# Autodesk Inventor assembly: Toughbox Nano Long Hex Output Shaft
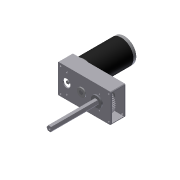
[picture p0: Inventor's stored thumbnail of the model, 180x180]
Saved by Autodesk Inventor 2013 (Build 170138000, 138)
## iProperties
Created: 2012-06-03
Part Number: Toughbox Nano Long Hex Output Shaft
Document SubType Name: Assembly
Designer: Nemo
Author: Nemo
## Documents named in this file (13)
- H:\Nemo\Documents\Robotics\COTS Parts\Gearboxes\Toughbox Nano Long Hex Output Shaft.iam
- H:\Nemo\Documents\Robotics\COTS Parts\Gearboxes\Components\AndyMark Housings\Toughbox Nano Tube Housing.ipt
- H:\Nemo\Documents\Robotics\COTS Parts\Gearboxes\Components\AndyMark Shafts\Toughbox Nano cluster shaft.ipt
- H:\Nemo\Documents\Robotics\COTS Parts\Bearings - AndyMark\Bearing FR6zz.ipt
- H:\Nemo\Documents\Robotics\COTS Parts\Bearings - AndyMark\Bearing FR6.ipt
- H:\Nemo\Documents\Robotics\COTS Parts\Bearings - AndyMark\Bearing FR6zz-hex.ipt
- H:\Nemo\Documents\Robotics\COTS Parts\Motors\Motor and Pinion Gear Assemblies\CIM Motor 14T.iam
- H:\Nemo\Documents\Robotics\COTS Parts\Bearings - AndyMark\Bearing FR8zz-hex.ipt
- H:\Nemo\Documents\Robotics\COTS Parts\Gearboxes\Components\AndyMark Shafts\Toughbox Long Hex Output Shaft.ipt
- H:\Nemo\Documents\Robotics\COTS Parts\Gears - AndyMark\Gear 20dp 375hex 50T.ipt
- H:\Nemo\Documents\Robotics\COTS Parts\Gears - AndyMark\Gear 20dp 375hex 14T.ipt
- H:\Nemo\Documents\Robotics\COTS Parts\Fasteners\e-klip 500.ipt
- H:\Nemo\Documents\Robotics\COTS Parts\Gears - AndyMark\Gear 20dp 500hex 50T.ipt
## Components (12 placed, 12 different names)
1. Toughbox Nano Tube Housing:1 — Insert:1, Insert:5, Insert:6, Insert:7, Insert:9, Mate:1, Mate:2, Mate:4, Mate:8, Mate:9
2. Toughbox Nano cluster shaft:1 — Insert:4, Angle:1, Angle:2, Angle:3
3. Bearing FR6zz:2 — Insert:1, Insert:8
4. Bearing FR6:1 — Insert:4, Insert:5, Mate:3
5. Bearing FR6zz-hex:1 — Angle:1, Insert:6, Mate:5
6. CIM Motor 14T:1 [sub-assembly] — Insert:9, Mate:1
7. Bearing FR8zz-hex:1 — Insert:7
8. Toughbox Long Hex Output Shaft:1 — Insert:8, Mate:6, Mate:7, Angle:4
9. Gear 20dp 375hex 50T:1 — Mate:2, Angle:2, Mate:3
10. Gear 14T 20dp 375hex:1 — Mate:4, Angle:3, Mate:5
11. e-klip 500:1 — Mate:6, Mate:7
12. Gear 50T 20dp 500hex:1 — Mate:8, Angle:4, Mate:9
## Relationships (20: Mate 9, Insert 7, Angle 4)
- Insert:1: Toughbox Nano Tube Housing:1 ↔ Bearing FR6zz:2
- Insert:4: Toughbox Nano cluster shaft:1 ↔ Bearing FR6:1
- Insert:5: Toughbox Nano Tube Housing:1 ↔ Bearing FR6:1
- Angle:1 (0 deg): Toughbox Nano cluster shaft:1 ↔ Bearing FR6zz-hex:1
- Insert:6: Toughbox Nano Tube Housing:1 ↔ Bearing FR6zz-hex:1
- Insert:7: Toughbox Nano Tube Housing:1 ↔ Bearing FR8zz-hex:1
- Insert:8: Bearing FR6zz:2 ↔ Toughbox Long Hex Output Shaft:1
- Insert:9: Toughbox Nano Tube Housing:1 ↔ CIM Motor 14T:1
- Mate:1: Toughbox Nano Tube Housing:1 ↔ CIM Motor 14T:1
- Mate:2: Toughbox Nano Tube Housing:1 ↔ Gear 20dp 375hex 50T:1
- Angle:2 (0 deg): Toughbox Nano cluster shaft:1 ↔ Gear 20dp 375hex 50T:1
- Mate:3: Bearing FR6:1 ↔ Gear 20dp 375hex 50T:1
- Mate:4: Toughbox Nano Tube Housing:1 ↔ Gear 14T 20dp 375hex:1
- Angle:3 (0 deg): Toughbox Nano cluster shaft:1 ↔ Gear 14T 20dp 375hex:1
- Mate:5: Bearing FR6zz-hex:1 ↔ Gear 14T 20dp 375hex:1
- Mate:6: Toughbox Long Hex Output Shaft:1 ↔ e-klip 500:1
- Mate:7 (0.254 mm): Toughbox Long Hex Output Shaft:1 ↔ e-klip 500:1
- Mate:8: Toughbox Nano Tube Housing:1 ↔ Gear 50T 20dp 500hex:1
- Angle:4 (0 deg): Toughbox Long Hex Output Shaft:1 ↔ Gear 50T 20dp 500hex:1
- Mate:9 (3.175 mm): Toughbox Nano Tube Housing:1 ↔ Gear 50T 20dp 500hex:1
